# Autodesk Inventor assembly: Assembly
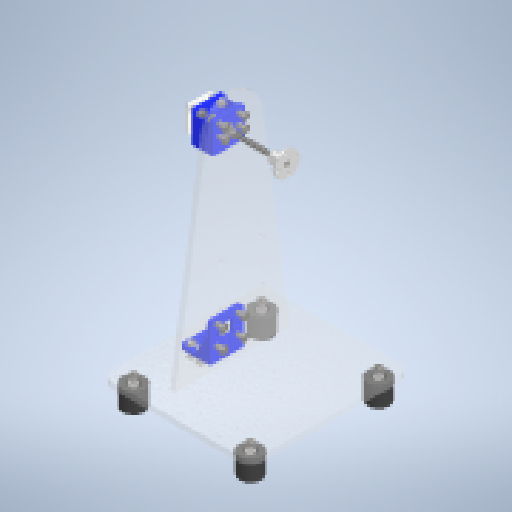
[picture p0: Inventor's stored thumbnail of the model, 512x512]
Saved by Autodesk Inventor 2023.1 (Build 271208000, 208)
## iProperties
Created: 2023-05-07
Part Number: Assembly
Document SubType Name: Assembly
Designer: felip
Author: felip
## Documents named in this file (15)
- C:\Users\felip\OneDrive\UNAL FORE\SEMESTRE 9\TECNICAS DE CONTROL\PROYECTO\PROYECTO-TDC-INVENTOR\Assembly - Fixed.iam
- C:\Users\felip\OneDrive\UNAL FORE\SEMESTRE 9\TECNICAS DE CONTROL\PROYECTO\PROYECTO-TDC-INVENTOR\base.ipt
- C:\Users\felip\OneDrive\UNAL FORE\SEMESTRE 9\TECNICAS DE CONTROL\PROYECTO\PROYECTO-TDC-INVENTOR\Pata-Goma.ipt
- C:\Users\felip\OneDrive\UNAL FORE\SEMESTRE 9\TECNICAS DE CONTROL\PROYECTO\PROYECTO-TDC-INVENTOR\BaseParal.ipt
- C:\Users\felip\OneDrive\UNAL FORE\SEMESTRE 9\TECNICAS DE CONTROL\PROYECTO\PROYECTO-TDC-INVENTOR\SoporteUnion.ipt
- C:\Users\felip\OneDrive\UNAL FORE\SEMESTRE 9\TECNICAS DE CONTROL\PROYECTO\PROYECTO-TDC-INVENTOR\SoporteEncoder.ipt
- C:\Users\felip\OneDrive\UNAL FORE\SEMESTRE 9\TECNICAS DE CONTROL\PROYECTO\PROYECTO-TDC-INVENTOR\rodamiento.ipt
- C:\Users\felip\OneDrive\UNAL FORE\SEMESTRE 9\TECNICAS DE CONTROL\PROYECTO\PROYECTO-TDC-INVENTOR\topito.ipt
- C:\Users\felip\OneDrive\UNAL FORE\SEMESTRE 9\TECNICAS DE CONTROL\PROYECTO\PROYECTO-TDC-INVENTOR\brida.ipt
- C:\Users\felip\OneDrive\UNAL FORE\SEMESTRE 9\TECNICAS DE CONTROL\PROYECTO\PROYECTO-TDC-INVENTOR\eje.ipt
- C:\Users\felip\OneDrive\UNAL FORE\SEMESTRE 9\TECNICAS DE CONTROL\PROYECTO\PROYECTO-TDC-INVENTOR\AS5600 v1.ipt
- C:\Users\felip\OneDrive\Documents\Inventor\Content Center Files\R2023\en-US\BS 4183(7)\BS 4183 - M3,5 x 8(2) III.ipt
- C:\Users\felip\OneDrive\Documents\Inventor\Content Center Files\R2023\en-US\BS 4183(4)\BS 4183 - M3,5 x 10(1) III.ipt
- C:\Users\felip\OneDrive\Documents\Inventor\Content Center Files\R2023\en-US\BS 4183(4)\BS 4183 - M2,5 x 14(1) III.ipt
- C:\Users\felip\OneDrive\Documents\Inventor\Content Center Files\R2023\en-US\BS 4183(1)\BS 4183 - M3,5(1).ipt
## Components (56 placed, 14 different names)
1. base:1 — Rotational:1, Rotational:2, Rotational:3, Rotational:4, Mate:1, Mate:2, Rotational:5, Rotational:6, Insert:4, Insert:5, Insert:6, Insert:7, Insert:39, Insert:40, Insert:41, Insert:42, Insert:43, Insert:44, Insert:45, Insert:46, Insert:60, Insert:61, Insert:62, Insert:63
2. Pata-Goma:1 — Rotational:1
3. Pata-Goma:2 — Rotational:2
4. Pata-Goma:3 — Rotational:3
5. Pata-Goma:4 — Rotational:4
6. BaseParal:1 — Mate:1, Mate:3, Rotational:7, Rotational:10, Rotational:11, Insert:47, Insert:48, Insert:49, Insert:50, Insert:51, Insert:52, Insert:53, Insert:54, Insert:55
7. SoporteUnion:1 — Mate:2, Rotational:5, Rotational:6, Mate:3, Rotational:7, Insert:8, Insert:10, Insert:11, Insert:12, Insert:13, Insert:15, Insert:17, Insert:18
8. SoporteEncoder:1 — Rotational:10, Rotational:11, Insert:1, Insert:2, Rotational:12, Rotational:13, Insert:29, Insert:30, Insert:31, Insert:33, Insert:67, Insert:68
9. rodamiento:1 — Insert:2, Rotational:14
10. rodamiento:2 — Insert:1
11. topito:1 — Rotational:12, Rotational:18
12. topito:2 — Rotational:13, Rotational:19
13. brida:1 — Insert:3
14. eje:1 — Rotational:14, Insert:3
15. AS5600 v1:1 — Rotational:18, Rotational:19, Insert:25, Insert:28
16. BS 4183 Slotted Pan Head Machine Screw - Metric M3,5 x 8:1 — Insert:4
17. BS 4183 Slotted Pan Head Machine Screw - Metric M3,5 x 8:2 — Insert:5
18. BS 4183 Slotted Pan Head Machine Screw - Metric M3,5 x 8:3 — Insert:6
19. BS 4183 Slotted Pan Head Machine Screw - Metric M3,5 x 8:4 — Insert:7
20. BS 4183 Specification for machine screws and machine screw nuts. Metric series - Metric M3,5 x 10:1 — Insert:8
21. BS 4183 Specification for machine screws and machine screw nuts. Metric series - Metric M3,5 x 10:3 — Insert:10
22. BS 4183 Specification for machine screws and machine screw nuts. Metric series - Metric M3,5 x 10:4 — Insert:11
23. BS 4183 Specification for machine screws and machine screw nuts. Metric series - Metric M3,5 x 10:5 — Insert:12
24. BS 4183 Specification for machine screws and machine screw nuts. Metric series - Metric M3,5 x 10:6 — Insert:13
25. BS 4183 Specification for machine screws and machine screw nuts. Metric series - Metric M3,5 x 10:8 — Insert:15
26. BS 4183 Specification for machine screws and machine screw nuts. Metric series - Metric M3,5 x 10:10 — Insert:17
27. BS 4183 Specification for machine screws and machine screw nuts. Metric series - Metric M3,5 x 10:11 — Insert:18
28. BS 4183 Specification for machine screws and machine screw nuts. Metric series - Metric M2,5 x 14:1 — Insert:25
29. BS 4183 Specification for machine screws and machine screw nuts. Metric series - Metric M2,5 x 14:4 — Insert:28
30. BS 4183 Specification for machine screws and machine screw nuts. Metric series - Metric M3,5 x 10:14 — Insert:29
31. BS 4183 Specification for machine screws and machine screw nuts. Metric series - Metric M3,5 x 10:15 — Insert:30
32. BS 4183 Specification for machine screws and machine screw nuts. Metric series - Metric M3,5 x 10:16 — Insert:31
33. BS 4183 Specification for machine screws and machine screw nuts. Metric series - Metric M3,5 x 10:18 — Insert:33
34. BS 4183 - Metric M3,5:1 — Insert:39
35. BS 4183 - Metric M3,5:2 — Insert:40
36. BS 4183 - Metric M3,5:3 — Insert:41
37. BS 4183 - Metric M3,5:4 — Insert:42
38. BS 4183 - Metric M3,5:5 — Insert:43
39. BS 4183 - Metric M3,5:6 — Insert:44
40. BS 4183 - Metric M3,5:7 — Insert:45
41. BS 4183 - Metric M3,5:8 — Insert:46
42. BS 4183 - Metric M3,5:9 — Insert:47
43. BS 4183 - Metric M3,5:10 — Insert:48
44. BS 4183 - Metric M3,5:11 — Insert:49
45. BS 4183 - Metric M3,5:12 — Insert:50
46. BS 4183 - Metric M3,5:13 — Insert:51
47. BS 4183 - Metric M3,5:14 — Insert:52
48. BS 4183 - Metric M3,5:15 — Insert:53
49. BS 4183 - Metric M3,5:16 — Insert:54
50. BS 4183 - Metric M3,5:17 — Insert:55
51. BS 4183 - Metric M3,5:18 — Insert:60
52. BS 4183 - Metric M3,5:19 — Insert:61
53. BS 4183 - Metric M3,5:20 — Insert:62
54. BS 4183 - Metric M3,5:21 — Insert:63
55. BS 4183 - Metric M3,5:22 — Insert:67
56. BS 4183 - Metric M3,5:23 — Insert:68
## Relationships (61: Insert 44, RevoluteJoint 14, Mate 3)
- Rotational:1 [RevoluteJoint]: base:1 ↔ Pata-Goma:1
- Rotational:2 [RevoluteJoint]: base:1 ↔ Pata-Goma:2
- Rotational:3 [RevoluteJoint]: base:1 ↔ Pata-Goma:3
- Rotational:4 [RevoluteJoint]: base:1 ↔ Pata-Goma:4
- Mate:1: base:1 ↔ BaseParal:1
- Mate:2: base:1 ↔ SoporteUnion:1
- Rotational:5 [RevoluteJoint]: base:1 ↔ SoporteUnion:1
- Rotational:6 [RevoluteJoint]: base:1 ↔ SoporteUnion:1
- Mate:3: BaseParal:1 ↔ SoporteUnion:1
- Rotational:7 [RevoluteJoint]: BaseParal:1 ↔ SoporteUnion:1
- Rotational:10 [RevoluteJoint]: BaseParal:1 ↔ SoporteEncoder:1
- Rotational:11 [RevoluteJoint]: BaseParal:1 ↔ SoporteEncoder:1
- Insert:1: SoporteEncoder:1 ↔ rodamiento:2
- Insert:2: SoporteEncoder:1 ↔ rodamiento:1
- Rotational:12 [RevoluteJoint]: SoporteEncoder:1 ↔ topito:1
- Rotational:13 [RevoluteJoint]: SoporteEncoder:1 ↔ topito:2
- Rotational:14 [RevoluteJoint]: rodamiento:1 ↔ eje:1
- Insert:3: brida:1 ↔ eje:1
- Rotational:18 [RevoluteJoint]: topito:1 ↔ AS5600 v1:1
- Rotational:19 [RevoluteJoint]: topito:2 ↔ AS5600 v1:1
- Insert:4: base:1 ↔ BS 4183 Slotted Pan Head Machine Screw - Metric M3,5 x 8:1
- Insert:5: base:1 ↔ BS 4183 Slotted Pan Head Machine Screw - Metric M3,5 x 8:2
- Insert:6: base:1 ↔ BS 4183 Slotted Pan Head Machine Screw - Metric M3,5 x 8:3
- Insert:7: base:1 ↔ BS 4183 Slotted Pan Head Machine Screw - Metric M3,5 x 8:4
- Insert:8: SoporteUnion:1 ↔ BS 4183 Specification for machine screws and machine screw nuts. Metric series - Metric M3,5 x 10:1
- Insert:10: SoporteUnion:1 ↔ BS 4183 Specification for machine screws and machine screw nuts. Metric series - Metric M3,5 x 10:3
- Insert:11: SoporteUnion:1 ↔ BS 4183 Specification for machine screws and machine screw nuts. Metric series - Metric M3,5 x 10:4
- Insert:12: SoporteUnion:1 ↔ BS 4183 Specification for machine screws and machine screw nuts. Metric series - Metric M3,5 x 10:5
- Insert:13: SoporteUnion:1 ↔ BS 4183 Specification for machine screws and machine screw nuts. Metric series - Metric M3,5 x 10:6
- Insert:15: SoporteUnion:1 ↔ BS 4183 Specification for machine screws and machine screw nuts. Metric series - Metric M3,5 x 10:8
- Insert:17: SoporteUnion:1 ↔ BS 4183 Specification for machine screws and machine screw nuts. Metric series - Metric M3,5 x 10:10
- Insert:18: SoporteUnion:1 ↔ BS 4183 Specification for machine screws and machine screw nuts. Metric series - Metric M3,5 x 10:11
- Insert:25: AS5600 v1:1 ↔ BS 4183 Specification for machine screws and machine screw nuts. Metric series - Metric M2,5 x 14:1
- Insert:28: AS5600 v1:1 ↔ BS 4183 Specification for machine screws and machine screw nuts. Metric series - Metric M2,5 x 14:4
- Insert:29: SoporteEncoder:1 ↔ BS 4183 Specification for machine screws and machine screw nuts. Metric series - Metric M3,5 x 10:14
- Insert:30: SoporteEncoder:1 ↔ BS 4183 Specification for machine screws and machine screw nuts. Metric series - Metric M3,5 x 10:15
- Insert:31: SoporteEncoder:1 ↔ BS 4183 Specification for machine screws and machine screw nuts. Metric series - Metric M3,5 x 10:16
- Insert:33: SoporteEncoder:1 ↔ BS 4183 Specification for machine screws and machine screw nuts. Metric series - Metric M3,5 x 10:18
- Insert:39: base:1 ↔ BS 4183 - Metric M3,5:1
- Insert:40: base:1 ↔ BS 4183 - Metric M3,5:2
- Insert:41: base:1 ↔ BS 4183 - Metric M3,5:3
- Insert:42: base:1 ↔ BS 4183 - Metric M3,5:4
- Insert:43: base:1 ↔ BS 4183 - Metric M3,5:5
- Insert:44: base:1 ↔ BS 4183 - Metric M3,5:6
- Insert:45: base:1 ↔ BS 4183 - Metric M3,5:7
- Insert:46: base:1 ↔ BS 4183 - Metric M3,5:8
- Insert:47: BaseParal:1 ↔ BS 4183 - Metric M3,5:9
- Insert:48: BaseParal:1 ↔ BS 4183 - Metric M3,5:10
- Insert:49: BaseParal:1 ↔ BS 4183 - Metric M3,5:11
- Insert:50: BaseParal:1 ↔ BS 4183 - Metric M3,5:12
- Insert:51: BaseParal:1 ↔ BS 4183 - Metric M3,5:13
- Insert:52: BaseParal:1 ↔ BS 4183 - Metric M3,5:14
- Insert:53: BaseParal:1 ↔ BS 4183 - Metric M3,5:15
- Insert:54: BaseParal:1 ↔ BS 4183 - Metric M3,5:16
- Insert:55: BaseParal:1 ↔ BS 4183 - Metric M3,5:17
- Insert:60: base:1 ↔ BS 4183 - Metric M3,5:18
- Insert:61: base:1 ↔ BS 4183 - Metric M3,5:19
- Insert:62: base:1 ↔ BS 4183 - Metric M3,5:20
- Insert:63: base:1 ↔ BS 4183 - Metric M3,5:21
- Insert:67: SoporteEncoder:1 ↔ BS 4183 - Metric M3,5:22
- Insert:68: SoporteEncoder:1 ↔ BS 4183 - Metric M3,5:23
